# Autodesk Inventor assembly: Ensamble_Pierna_delantera
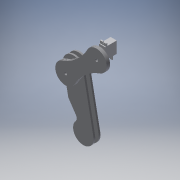
[picture p0: Inventor's stored thumbnail of the model, 180x180]
Saved by Autodesk Inventor 2019 (Build 230136000, 136)
## iProperties
Created: 2020-02-12
Part Number: Ensamble_Pierna_delantera
Document SubType Name: Assembly
Designer: jacqu
Author: jacqu
## Documents named in this file (5)
- C:\Users\Mafer1\Desktop\UVG\S9\Robotica\ProyectoCuadrupedo\Proyecto1\Proyecto1\Ensamble_Pierna_delantera.iam
- C:\Users\Mafer1\Desktop\UVG\S9\Robotica\ProyectoCuadrupedo\Proyecto1\Proyecto1\pierna1.ipt
- C:\Users\Mafer1\Desktop\UVG\S9\Robotica\ProyectoCuadrupedo\Proyecto1\Proyecto1\pierna1_2.ipt
- C:\Users\Mafer1\Desktop\UVG\S9\Robotica\ProyectoCuadrupedo\Proyecto1\Proyecto1\Pierna2.ipt
- C:\Users\Mafer1\Desktop\UVG\S9\Robotica\ProyectoCuadrupedo\Proyecto1\Proyecto1\servo.ipt
## Components (6 placed, 4 different names)
1. pierna1:1 — Mate:4, Mate:5, Mate:6
2. pierna1_2:1 — Mate:4, Mate:5, Mate:6, Mate:12, Mate:13, Mate:14, Mate:15
3. Pierna2:1 — Mate:7, Mate:19, Mate:20
4. servo:1 — Mate:7, Mate:9, Mate:12, Mate:13, Mate:19, Mate:20, Mate:21, Mate:22
5. servo:2 — Mate:14, Mate:15
6. Pierna2:2 — Mate:9, Mate:21, Mate:22
## Relationships (13: Mate 13)
- Mate:4: pierna1:1 ↔ pierna1_2:1
- Mate:5: pierna1:1 ↔ pierna1_2:1
- Mate:6: pierna1:1 ↔ pierna1_2:1
- Mate:7: Pierna2:1 ↔ servo:1
- Mate:9: servo:1 ↔ Pierna2:2
- Mate:12: pierna1_2:1 ↔ servo:1
- Mate:13: pierna1_2:1 ↔ servo:1
- Mate:14: pierna1_2:1 ↔ servo:2
- Mate:15: pierna1_2:1 ↔ servo:2
- Mate:19: Pierna2:1 ↔ servo:1
- Mate:20: Pierna2:1 ↔ servo:1
- Mate:21: servo:1 ↔ Pierna2:2
- Mate:22: servo:1 ↔ Pierna2:2
